# Autodesk Inventor assembly: Rack and pinion
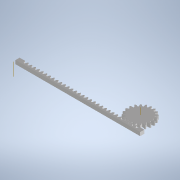
[picture p0: Inventor's stored thumbnail of the model, 180x180]
Saved by Autodesk Inventor 2020 (Build 240168000, 168)
## iProperties
Created: 2021-01-11
Part Number: Rack and pinion
Document SubType Name: Assembly
Designer: moham
Author: moham
## Documents named in this file (3)
- D:\Projects\MCT 131\The project\Lifter\Rack and pinion.iam
- D:\Projects\MCT 131\The project\Lifter\Pinion_4.ipt
- D:\Projects\MCT 131\The project\Lifter\Rack_4.ipt
## Components (2 placed, 2 different names)
1. Pinion_4:1 — Mate:1, Flush:1, Flush:2, Rotation/Translation:1
2. Rack_4:1 — Flush:2, Flush:3, Rotation/Translation:1
## Relationships (5: Flush 3, Mate 1, RelateRotateTranslate 1)
- Mate:1: Pinion_4:1
- Flush:1: Pinion_4:1
- Flush:2: Pinion_4:1 ↔ Rack_4:1
- Flush:3 (20 mm): Rack_4:1
- Rotation/Translation:1 [RelateRotateTranslate] (125.6637 mm): Pinion_4:1 ↔ Rack_4:1
